# Autodesk Inventor assembly: ONDERPLAAT
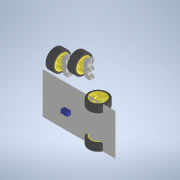
[picture p0: Inventor's stored thumbnail of the model, 180x180]
Saved by Autodesk Inventor 2022 (Build 260153000, 153)
## iProperties
Created: 2021-12-16
Part Number: ONDERPLAAT
Document SubType Name: Assembly
Designer: keemi
Author: keemi
## Documents named in this file (6)
- C:\Users\keemi\OneDrive\Bureaublad\repo's\projecten\Auto\modellen\inventor\auto moddel\ONDERPLAAT.iam
- C:\Users\keemi\OneDrive\Bureaublad\repo's\projecten\Auto\modellen\inventor\auto moddel\onderkant.ipt
- C:\Users\keemi\OneDrive\Bureaublad\repo's\projecten\Auto\modellen\inventor\geared-dc-motor-for-arduino-applications-1.snapshot.2\Hobi - Motor DC 1.ipt
- C:\Users\keemi\OneDrive\Bureaublad\repo's\projecten\Auto\modellen\inventor\wheel-arduino-1.snapshot.2\Wheel ALL.ipt
- C:\Users\keemi\OneDrive\Bureaublad\repo's\projecten\Auto\modellen\inventor\auto moddel\VOORWIEL_TOTAAL.iam
- C:\Users\keemi\OneDrive\Bureaublad\repo's\projecten\Auto\modellen\inventor\SG90\SG90 v1.ipt
## Components (8 placed, 5 different names)
1. onderkant:1 — Mate:9, Flush:1, Mate:10, Flush:3, Flush:4, Mate:11, Flush:5
2. Hobi - Motor DC 1:1 — Mate:1, Mate:2, Mate:10, Flush:2, Flush:4
3. Wheel ALL:1 — Mate:1, Mate:2
4. Hobi - Motor DC 1:2 — Mate:9, Flush:1, Flush:2, Flush:3
5. Wheel ALL:2
6. VOORWIEL_TOTAAL:1 [sub-assembly]
7. VOORWIEL_TOTAAL:2 [sub-assembly]
8. SG90 v1:1 — Mate:11, Flush:5
## Relationships (12: Mate 7, Flush 5)
- Mate:1: Hobi - Motor DC 1:1 ↔ Wheel ALL:1
- Mate:2: Hobi - Motor DC 1:1 ↔ Wheel ALL:1
- [Mate]: Hobi - Motor DC 1:2 ↔ Wheel ALL:2
- [Mate]: Hobi - Motor DC 1:2 ↔ Wheel ALL:2
- Mate:9: onderkant:1 ↔ Hobi - Motor DC 1:2
- Flush:1 (70 mm): onderkant:1 ↔ Hobi - Motor DC 1:2
- Mate:10: onderkant:1 ↔ Hobi - Motor DC 1:1
- Flush:2: Hobi - Motor DC 1:1 ↔ Hobi - Motor DC 1:2
- Flush:3 (30 mm): onderkant:1 ↔ Hobi - Motor DC 1:2
- Flush:4 (30 mm): onderkant:1 ↔ Hobi - Motor DC 1:1
- Mate:11: onderkant:1 ↔ SG90 v1:1
- Flush:5 (70 mm): onderkant:1 ↔ SG90 v1:1
## Named parameters: d2_d0 = 0 mm, d3_d1 = 0 mm
